# Autodesk Inventor assembly: Редуктор
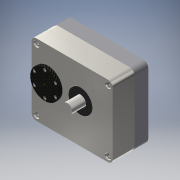
[picture p0: Inventor's stored thumbnail of the model, 180x180]
Saved by Autodesk Inventor 2016 (Build 200138000, 138)
## iProperties
Created: 2021-04-28
Part Number: Редуктор
Material: Типовые
Document SubType Name: Assembly
Designer: Лол
Author: Лол
## Documents named in this file (23)
- C:\Users\Лол\Documents\Inventor\course_work\Редуктор.iam
- C:\Users\Лол\Documents\Inventor\course_work\Корпус часть без резьбы.ipt
- C:\Users\Лол\Documents\Inventor\course_work\Подшипник\Подшипник-01.ipt
- C:\Users\Лол\Documents\Inventor\course_work\Подшипник.ipt
- C:\Users\Лол\Documents\Inventor\course_work\Подшипник\Подшипник-02.ipt
- C:\Users\Лол\Documents\Inventor\course_work\Быстроходный вал.ipt
- C:\Users\Лол\Documents\Inventor\course_work\Тихоходный вал.ipt
- C:\Users\Лол\Documents\Inventor\course_work\Кольцо A30 ГОСТ 13942-86.ipt
- C:\Users\Лол\Documents\Inventor\course_work\Кольцо A35 ГОСТ 13942-86.ipt
- C:\Users\Лол\Documents\Inventor\course_work\Быстроходое колесо.ipt
- C:\Users\Лол\Documents\Inventor\course_work\Корпус центральная часть.ipt
- C:\Users\Лол\Documents\Inventor\course_work\Корпус часть с резьбой.ipt
- C:\Users\Лол\Documents\Inventor\course_work\Гайка M30x1.5 6H ГОСТ 6393-73.ipt
- C:\Users\Лол\Documents\Inventor\course_work\Гайка M33x1.5 6H ГОСТ 6393-73.ipt
- C:\Users\Лол\Documents\Inventor\course_work\ISO 2340 - A - 6 x 40ISO.ipt
- C:\Users\Лол\Documents\Inventor\course_work\AS 1420 - 1973 - M10 x 75.ipt
- C:\Users\Лол\Documents\Inventor\course_work\Крышка маленькая_62.ipt
- C:\Users\Лол\Documents\Inventor\course_work\КОЛЬЦО 062-066-25 гост 9833.ipt
- C:\Users\Лол\Documents\Inventor\course_work\Манжет 1-30x72x10 ГОСТ 8752-79.ipt
- C:\Users\Лол\Documents\Inventor\course_work\Манжет 1-28x62x10 ГОСТ 8752-79.ipt
- C:\Users\Лол\Documents\Inventor\course_work\Крышка большая_72.ipt
- C:\Users\Лол\Documents\Inventor\course_work\КОЛЬЦО 072-066-25 гост 9833.ipt
- C:\Users\Лол\Documents\Inventor\course_work\AS 1420 - 1973 - M6 x 12.ipt
## Components (38 placed, 21 different names)
1. Корпус часть без резьбы:1 — Заподлицо:1, Заподлицо:2, Заподлицо:3, Совмещение:1, Совмещение:2, Совмещение:3, Совмещение:4, Совмещение:14, Совмещение:27, Совмещение:28, Совмещение:33, Совмещение:34, Совмещение:35, Совмещение:36, Совмещение:37, Совмещение:38, Совмещение:39, Совмещение:40, Совмещение:43, Совмещение:44, Совмещение:46, Заподлицо:4, Совмещение:61, Совмещение:62
2. Подшипник-01:1 — Совмещение:18, Совмещение:19, Совмещение:22, Совмещение:24
3. Подшипник-01:2 — Совмещение:1, Совмещение:2, Совмещение:5, Совмещение:13
4. Подшипник-02:3 — Совмещение:3, Совмещение:4, Совмещение:6, Совмещение:26
5. Подшипник-02:4 — Совмещение:16, Совмещение:17, Совмещение:, Совмещение:21
6. Быстроходный вал:1 — Совмещение:5, Совмещение:7, Совмещение:8, Совмещение:22, Совмещение:23
7. Тихоходный вал:1 — Совмещение:6, Совмещение:9, Совмещение:11, Совмещение:12, Совмещение:21, Совмещение:25, Совмещение:48, Совмещение:52
8. Кольцо A30 ГОСТ 13942-86:1 — Совмещение:7, Совмещение:8, Совмещение:13
9. Кольцо A35 ГОСТ 13942-86:1 — Совмещение:9, Совмещение:, Совмещение:48
10. Быстроходое колесо:2 — Совмещение:11, Совмещение:12, Совмещение:52
11. Корпус центральная часть:1 — Совмещение:14, Совмещение:15, Совмещение:29, Совмещение:30, Совмещение:31, Совмещение:32
12. Корпус часть с резьбой:1 — Совмещение:15, Совмещение:16, Совмещение:17, Совмещение:18, Совмещение:19, Совмещение:47, Заподлицо:5, Совмещение:49, Совмещение:56, Совмещение:57, Совмещение:65
13. Гайка M30x1.5 6H ГОСТ 6393-73:1 — Совмещение:23, Совмещение:24
14. Гайка M33x1.5 6H ГОСТ 6393-73:1 — Совмещение:25, Совмещение:26
15. ISO 2340 - A - 6 x 40ISO:1 — Совмещение:27, Совмещение:29, Совмещение:31
16. ISO 2340 - A - 6 x 40ISO:2 — Совмещение:28, Совмещение:30, Совмещение:32
17. AS 1420 - 1973 - M10 x 75:1 — Совмещение:33, Совмещение:34
18. AS 1420 - 1973 - M10 x 75:2 — Совмещение:35, Совмещение:36
19. AS 1420 - 1973 - M10 x 75:3 — Совмещение:37, Совмещение:38
20. AS 1420 - 1973 - M10 x 75:4 — Совмещение:39, Совмещение:40
21. Крышка маленькая_62:1 — Совмещение:41, Совмещение:42, Совмещение:43, Совмещение:44, Совмещение:61, Совмещение:63, Совмещение:64
22. КОЛЬЦО 062-066-25 гост 9833:1 — Совмещение:41, Совмещение:42
23. Манжет 1-30x72x10 ГОСТ 8752-79:2 — Совмещение:46, Заподлицо:4
24. Манжет 1-28x62x10 ГОСТ 8752-79:2 — Совмещение:47, Заподлицо:5
25. Крышка большая_72:2 — Совмещение:49, Совмещение:50, Совмещение:51, Совмещение:56, Совмещение:57, Совмещение:60, Совмещение:66
26. КОЛЬЦО 072-066-25 гост 9833:1 — Совмещение:50, Совмещение:51
27. AS 1420 - 1973 - M6 x 12:1 — Совмещение:62, Совмещение:63
28. AS 1420 - 1973 - M6 x 12:2
29. AS 1420 - 1973 - M6 x 12:3
30. AS 1420 - 1973 - M6 x 12:4
31. AS 1420 - 1973 - M6 x 12:5
32. AS 1420 - 1973 - M6 x 12:6
33. AS 1420 - 1973 - M6 x 12:8 — Совмещение:65, Совмещение:66
34. AS 1420 - 1973 - M6 x 12:9
35. AS 1420 - 1973 - M6 x 12:10
36. AS 1420 - 1973 - M6 x 12:11
37. AS 1420 - 1973 - M6 x 12:12
38. AS 1420 - 1973 - M6 x 12:13
## Component patterns: (6 elements, first: AS 1420 - 1973 - M6 x 12:1), (6 elements, first: AS 1420 - 1973 - M6 x 12:8)
## Relationships (64: Mate 59, Flush 5)
- Заподлицо:1 [Flush]: Корпус часть без резьбы:1
- Заподлицо:2 [Flush] (-37.142 mm): Корпус часть без резьбы:1
- Заподлицо:3 [Flush] (-27.571 mm): Корпус часть без резьбы:1
- Совмещение:1 [Mate]: Корпус часть без резьбы:1 ↔ Подшипник-01:2
- Совмещение:2 [Mate]: Корпус часть без резьбы:1 ↔ Подшипник-01:2
- Совмещение:3 [Mate]: Корпус часть без резьбы:1 ↔ Подшипник-02:3
- Совмещение:4 [Mate]: Корпус часть без резьбы:1 ↔ Подшипник-02:3
- Совмещение:5 [Mate]: Подшипник-01:2 ↔ Быстроходный вал:1
- Совмещение:6 [Mate]: Подшипник-02:3 ↔ Тихоходный вал:1
- Совмещение:7 [Mate]: Быстроходный вал:1 ↔ Кольцо A30 ГОСТ 13942-86:1
- Совмещение:8 [Mate]: Быстроходный вал:1 ↔ Кольцо A30 ГОСТ 13942-86:1
- Совмещение:9 [Mate]: Тихоходный вал:1 ↔ Кольцо A35 ГОСТ 13942-86:1
- Совмещение:11 [Mate]: Тихоходный вал:1 ↔ Быстроходое колесо:2
- Совмещение:12 [Mate]: Тихоходный вал:1 ↔ Быстроходое колесо:2
- Совмещение:13 [Mate]: Подшипник-01:2 ↔ Кольцо A30 ГОСТ 13942-86:1
- Совмещение:14 [Mate]: Корпус часть без резьбы:1 ↔ Корпус центральная часть:1
- Совмещение:15 [Mate]: Корпус центральная часть:1 ↔ Корпус часть с резьбой:1
- Совмещение:16 [Mate]: Подшипник-02:4 ↔ Корпус часть с резьбой:1
- Совмещение:17 [Mate]: Подшипник-02:4 ↔ Корпус часть с резьбой:1
- Совмещение:18 [Mate]: Подшипник-01:1 ↔ Корпус часть с резьбой:1
- Совмещение:19 [Mate]: Подшипник-01:1 ↔ Корпус часть с резьбой:1
- Совмещение: [Mate]: Подшипник-02:4 ↔ Кольцо A35 ГОСТ 13942-86:1
- Совмещение:21 [Mate]: Подшипник-02:4 ↔ Тихоходный вал:1
- Совмещение:22 [Mate]: Подшипник-01:1 ↔ Быстроходный вал:1
- Совмещение:23 [Mate]: Быстроходный вал:1 ↔ Гайка M30x1.5 6H ГОСТ 6393-73:1
- Совмещение:24 [Mate]: Подшипник-01:1 ↔ Гайка M30x1.5 6H ГОСТ 6393-73:1
- Совмещение:25 [Mate]: Тихоходный вал:1 ↔ Гайка M33x1.5 6H ГОСТ 6393-73:1
- Совмещение:26 [Mate]: Подшипник-02:3 ↔ Гайка M33x1.5 6H ГОСТ 6393-73:1
- Совмещение:27 [Mate]: Корпус часть без резьбы:1 ↔ ISO 2340 - A - 6 x 40ISO:1
- Совмещение:28 [Mate]: Корпус часть без резьбы:1 ↔ ISO 2340 - A - 6 x 40ISO:2
- Совмещение:29 [Mate]: Корпус центральная часть:1 ↔ ISO 2340 - A - 6 x 40ISO:1
- Совмещение:30 [Mate]: Корпус центральная часть:1 ↔ ISO 2340 - A - 6 x 40ISO:2
- Совмещение:31 [Mate] (7.5 mm): Корпус центральная часть:1 ↔ ISO 2340 - A - 6 x 40ISO:1
- Совмещение:32 [Mate] (7.5 mm): Корпус центральная часть:1 ↔ ISO 2340 - A - 6 x 40ISO:2
- Совмещение:33 [Mate]: Корпус часть без резьбы:1 ↔ AS 1420 - 1973 - M10 x 75:1
- Совмещение:34 [Mate]: Корпус часть без резьбы:1 ↔ AS 1420 - 1973 - M10 x 75:1
- Совмещение:35 [Mate]: Корпус часть без резьбы:1 ↔ AS 1420 - 1973 - M10 x 75:2
- Совмещение:36 [Mate]: Корпус часть без резьбы:1 ↔ AS 1420 - 1973 - M10 x 75:2
- Совмещение:37 [Mate]: Корпус часть без резьбы:1 ↔ AS 1420 - 1973 - M10 x 75:3
- Совмещение:38 [Mate]: Корпус часть без резьбы:1 ↔ AS 1420 - 1973 - M10 x 75:3
- Совмещение:39 [Mate]: Корпус часть без резьбы:1 ↔ AS 1420 - 1973 - M10 x 75:4
- Совмещение:40 [Mate]: Корпус часть без резьбы:1 ↔ AS 1420 - 1973 - M10 x 75:4
- Совмещение:41 [Mate]: Крышка маленькая_62:1 ↔ КОЛЬЦО 062-066-25 гост 9833:1
- Совмещение:42 [Mate] (1.25 mm): Крышка маленькая_62:1 ↔ КОЛЬЦО 062-066-25 гост 9833:1
- Совмещение:43 [Mate]: Корпус часть без резьбы:1 ↔ Крышка маленькая_62:1
- Совмещение:44 [Mate]: Корпус часть без резьбы:1 ↔ Крышка маленькая_62:1
- Совмещение:46 [Mate]: Корпус часть без резьбы:1 ↔ Манжет 1-30x72x10 ГОСТ 8752-79:2
- Заподлицо:4 [Flush]: Корпус часть без резьбы:1 ↔ Манжет 1-30x72x10 ГОСТ 8752-79:2
- Совмещение:47 [Mate]: Корпус часть с резьбой:1 ↔ Манжет 1-28x62x10 ГОСТ 8752-79:2
- Заподлицо:5 [Flush]: Корпус часть с резьбой:1 ↔ Манжет 1-28x62x10 ГОСТ 8752-79:2
- Совмещение:48 [Mate]: Тихоходный вал:1 ↔ Кольцо A35 ГОСТ 13942-86:1
- Совмещение:49 [Mate]: Корпус часть с резьбой:1 ↔ Крышка большая_72:2
- Совмещение:50 [Mate]: Крышка большая_72:2 ↔ КОЛЬЦО 072-066-25 гост 9833:1
- Совмещение:51 [Mate] (1.25 mm): Крышка большая_72:2 ↔ КОЛЬЦО 072-066-25 гост 9833:1
- Совмещение:52 [Mate]: Тихоходный вал:1 ↔ Быстроходое колесо:2
- Совмещение:56 [Mate]: Корпус часть с резьбой:1 ↔ Крышка большая_72:2
- Совмещение:57 [Mate]: Корпус часть с резьбой:1 ↔ Крышка большая_72:2
- Совмещение:60 [Mate]: Крышка большая_72:2
- Совмещение:61 [Mate]: Корпус часть без резьбы:1 ↔ Крышка маленькая_62:1
- Совмещение:62 [Mate]: Корпус часть без резьбы:1 ↔ AS 1420 - 1973 - M6 x 12:1
- Совмещение:63 [Mate]: Крышка маленькая_62:1 ↔ AS 1420 - 1973 - M6 x 12:1
- Совмещение:64 [Mate]: Крышка маленькая_62:1
- Совмещение:65 [Mate]: Корпус часть с резьбой:1 ↔ AS 1420 - 1973 - M6 x 12:8
- Совмещение:66 [Mate]: Крышка большая_72:2 ↔ AS 1420 - 1973 - M6 x 12:8
